# Autodesk Inventor assembly: Hexapod
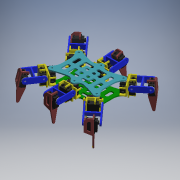
[picture p0: Inventor's stored thumbnail of the model, 180x180]
Saved by Autodesk Inventor 2017 (Build 210142000, 142)
## iProperties
Part Number: Hexapod
Document SubType Name: Assembly
Designer: Alexander Miller
Author: Alexander Miller
## Documents named in this file (9)
- D:\Daten\Documents\Git\Hexapod\3DParts\Hexapod.iam
- D:\Daten\Documents\Git\Hexapod\3DParts\Body_bottom.ipt
- D:\Daten\Documents\Git\Hexapod\3DParts\leg_right.iam
- D:\Daten\Documents\Git\Hexapod\3DParts\Body_top.ipt
- D:\Daten\Documents\Git\Hexapod\3DParts\Servo.ipt
- D:\Daten\Documents\Git\Hexapod\3DParts\Servo_arm.ipt
- D:\Daten\Documents\Git\Hexapod\3DParts\ball_bearing.ipt
- D:\Daten\Documents\Git\Hexapod\3DParts\leg_left.iam
- D:\Daten\Documents\Git\Hexapod\3DParts\Connector.ipt
## Components (20 placed, 6 different names)
1. leg_right:1 [sub-assembly] — Rigid:3, Rigid:16
2. leg_right:2 [sub-assembly] — Rigid:4, Rigid:17
3. leg_right:3 [sub-assembly] — Rigid:2, Rigid:18
4. Body_top:1 — Rigid:2, Rigid:3, Rigid:4, Mate:1, Flush:1, Flush:2, Rigid:13, Rigid:14, Rigid:15
5. Body_bottom:1 — Mate:1, Flush:1, Flush:2, Rigid:7, Rigid:8, Rigid:9, Rigid:10, Rigid:11, Rigid:12
6. ball_bearing:1 — Rigid:7
7. ball_bearing:2 — Rigid:12
8. ball_bearing:3 — Rigid:11
9. ball_bearing:4 — Rigid:8
10. ball_bearing:5 — Rigid:10
11. ball_bearing:6 — Rigid:9
12. leg_left:1 [sub-assembly] — Rigid:13, Rigid:19
13. leg_left:2 [sub-assembly] — Rigid:14, Rigid:20
14. leg_left:3 [sub-assembly] — Rigid:15, Rigid:21
15. Connector:1 — Rigid:16
16. Connector:2 — Rigid:17
17. Connector:3 — Rigid:18
18. Connector:4 — Rigid:19
19. Connector:5 — Rigid:20
20. Connector:6 — Rigid:21
## Relationships (21: WeldJoint 18, Flush 2, Mate 1)
- Rigid:2 [WeldJoint]: leg_right:3 ↔ Body_top:1
- Rigid:3 [WeldJoint]: leg_right:1 ↔ Body_top:1
- Rigid:4 [WeldJoint]: leg_right:2 ↔ Body_top:1
- Mate:1 (51 mm): Body_top:1 ↔ Body_bottom:1
- Flush:1: Body_top:1 ↔ Body_bottom:1
- Flush:2: Body_top:1 ↔ Body_bottom:1
- Rigid:7 [WeldJoint]: Body_bottom:1 ↔ ball_bearing:1
- Rigid:8 [WeldJoint]: Body_bottom:1 ↔ ball_bearing:4
- Rigid:9 [WeldJoint]: Body_bottom:1 ↔ ball_bearing:6
- Rigid:10 [WeldJoint]: Body_bottom:1 ↔ ball_bearing:5
- Rigid:11 [WeldJoint]: Body_bottom:1 ↔ ball_bearing:3
- Rigid:12 [WeldJoint]: Body_bottom:1 ↔ ball_bearing:2
- Rigid:13 [WeldJoint]: Body_top:1 ↔ leg_left:1
- Rigid:14 [WeldJoint]: Body_top:1 ↔ leg_left:2
- Rigid:15 [WeldJoint]: Body_top:1 ↔ leg_left:3
- Rigid:16 [WeldJoint]: leg_right:1 ↔ Connector:1
- Rigid:17 [WeldJoint]: leg_right:2 ↔ Connector:2
- Rigid:18 [WeldJoint]: leg_right:3 ↔ Connector:3
- Rigid:19 [WeldJoint]: leg_left:1 ↔ Connector:4
- Rigid:20 [WeldJoint]: leg_left:2 ↔ Connector:5
- Rigid:21 [WeldJoint]: leg_left:3 ↔ Connector:6
## Named parameters: b_mat_thickness = 5 mm, s_height = 38 mm, s_shaft_height = 6 mm, sa_thickness = 2 mm
